# Autodesk Inventor assembly: Total assembly
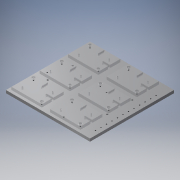
[picture p0: Inventor's stored thumbnail of the model, 180x180]
Saved by Autodesk Inventor 2017 (Build 210142000, 142)
## iProperties
Created: 2016-09-16
Part Number: Total assembly
Document SubType Name: Assembly
Designer: Andreas Fröderberg
Author: Andreas Fröderberg
## Documents named in this file (3)
- C:\Users\Andreas Fröderberg\Documents\Inventor\PCB Fixture\Total assembly.iam
- C:\Users\Andreas Fröderberg\Documents\Inventor\PCB Fixture\Base plate.ipt
- C:\Users\Andreas Fröderberg\Documents\Inventor\PCB Fixture\PCB FIxture 80x50.ipt
## Components (7 placed, 2 different names)
1. Base plate:1 — Mate:1, Mate:2, Mate:3, Mate:4, Mate:5, Mate:6
2. PCB FIxture 80x50:1 — Mate:1
3. PCB FIxture 80x50:2 — Mate:2
4. PCB FIxture 80x50:3 — Mate:3
5. PCB FIxture 80x50:4 — Mate:4
6. PCB FIxture 80x50:5 — Mate:5
7. PCB FIxture 80x50:6 — Mate:6
## Relationships (6: Mate 6)
- Mate:1: Base plate:1 ↔ PCB FIxture 80x50:1
- Mate:2: Base plate:1 ↔ PCB FIxture 80x50:2
- Mate:3: Base plate:1 ↔ PCB FIxture 80x50:3
- Mate:4: Base plate:1 ↔ PCB FIxture 80x50:4
- Mate:5: Base plate:1 ↔ PCB FIxture 80x50:5
- Mate:6: Base plate:1 ↔ PCB FIxture 80x50:6
